# Autodesk Inventor assembly: Main Assembly
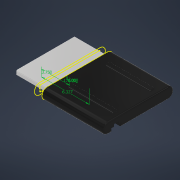
[picture p0: Inventor's stored thumbnail of the model, 180x180]
Saved by Autodesk Inventor 2021.3 (Build 253353000, 353)
## iProperties
Created: 2021-06-17
Part Number: Main Assembly
Document SubType Name: Assembly
Designer: trl121
Author: trl121
## Documents named in this file (4)
- D:\trl121\Documents\_repositories\RazerBook13Dock\Inventor\Main Assembly.iam
- D:\trl121\Documents\_repositories\RazerBook13Dock\Inventor\Razor Book 13.ipt
- D:\trl121\Documents\_repositories\RazerBook13Dock\Inventor\Bottom Part.ipt
- D:\trl121\Documents\_repositories\RazerBook13Dock\Inventor\Top Part.ipt
## Components (3 placed, 3 different names)
1. Razor Book 13:1 — Flush:1
2. Bottom Part:1 — Flush:1, Flush:2, Flush:6, Flush:10
3. Top Part:1 — Flush:2, Flush:6, Flush:10
## Relationships (4: Flush 4)
- Flush:1: Razor Book 13:1 ↔ Bottom Part:1
- Flush:2: Bottom Part:1 ↔ Top Part:1
- Flush:6: Bottom Part:1 ↔ Top Part:1
- Flush:10: Bottom Part:1 ↔ Top Part:1
